# Autodesk Inventor assembly: pulley thing assmble
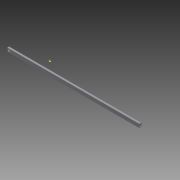
[picture p0: Inventor's stored thumbnail of the model, 180x180]
Saved by Autodesk Inventor 2015 (Build 190159000, 159)
## iProperties
Created: 2015-01-17
Part Number: pulley thing assmble
Document SubType Name: Assembly
Designer: whitaus15
Author: whitaus15
## Documents named in this file (3)
- \\lhssvr02\Homedirs\Robotics Club\Hardware\CAD\claw\pulley thing assmble.iam
- \\lhssvr02\Homedirs\Robotics Club\Hardware\CAD\claw\box beam.ipt
- \\lhssvr02\Homedirs\Robotics Club\Hardware\CAD\claw\hexagon bearing.ipt
## Components (3 placed, 2 different names)
1. box beam:2 — Mate:1
2. hexagon bearing:1 — Mate:1
3. hexagon bearing:2
## Relationships (1: Mate 1)
- Mate:1: box beam:2 ↔ hexagon bearing:1
